# Autodesk Inventor assembly: ENSAMBLE_NUEVA_CREMALLERA
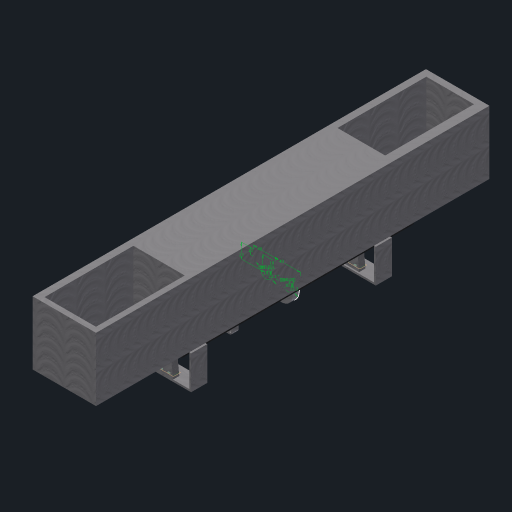
[picture p0: Inventor's stored thumbnail of the model, 512x512]
Saved by Autodesk Inventor 2024.3 (Build 283343000, 343)
## iProperties
Created: 2024-08-24
Part Number: ENSAMBLE_NUEVA_CREMALLERA
Material: Generic
Document SubType Name: Assembly
Designer: Niler
Author: Niler
## Documents named in this file (11)
- C:\Users\Niler\OneDrive\Escritorio\RECICLADOR\RECICLADOR_MODELO_3D\NUEVA CREMALLERA\ENSAMBLE_NUEVA_CREMALLERA.iam
- C:\Users\Niler\OneDrive\Escritorio\RECICLADOR\RECICLADOR_MODELO_3D\NUEVA CREMALLERA\TUBO.ipt
- C:\Users\Niler\OneDrive\Escritorio\RECICLADOR\RECICLADOR_MODELO_3D\NUEVA CREMALLERA\DESLIZANTE.ipt
- C:\Users\Niler\OneDrive\Escritorio\RECICLADOR\RECICLADOR_MODELO_3D\NUEVA CREMALLERA\APOYO_PLETINA.ipt
- C:\Users\Niler\OneDrive\Escritorio\RECICLADOR\RECICLADOR_MODELO_3D\NUEVA CREMALLERA\PARA_TUERCA.ipt
- C:\Users\Niler\OneDrive\Escritorio\RECICLADOR\RECICLADOR_MODELO_3D\NUEVA CREMALLERA\OTRO_EXTREMO.ipt
- C:\Users\Niler\OneDrive\Escritorio\RECICLADOR\RECICLADOR_MODELO_3D\NUEVA CREMALLERA\TORNILLO.ipt
- C:\Users\Niler\OneDrive\Escritorio\RECICLADOR\RECICLADOR_MODELO_3D\NUEVA CREMALLERA\GUIA.ipt
- C:\Users\Niler\OneDrive\Escritorio\RECICLADOR\RECICLADOR_MODELO_3D\MECANISMO DE COMPACTADO\NEMA 17 PARA TAPA PRINCIPAL.ipt
- C:\Users\Niler\OneDrive\Escritorio\RECICLADOR\RECICLADOR_MODELO_3D\MECANISMO DE COMPACTADO\ACOPLE_NEMA_PUERTA.ipt
- C:\Users\Niler\OneDrive\Escritorio\RECICLADOR\RECICLADOR_MODELO_3D\NUEVA CREMALLERA\PARA_TUERCA_V2.ipt
## Components (14 placed, 10 different names)
1. TUBO:1 — Flush:1, Mate:1, Mate:2, Mate:3, Mate:4, Mate:5
2. DESLIZANTE:1 — Flush:1, Mate:1, Flush:2, Mate:6, Mate:17
3. APOYO_PLETINA:1 — Mate:2, Mate:3, Mate:7, Flush:4, Mate:12, Flush:6, Mate:15
4. APOYO_PLETINA:2 — Mate:4, Mate:5, Mate:13
5. PARA_TUERCA:1 — Flush:2, Mate:6, Mate:8, Flush:5
6. OTRO_EXTREMO:1 — Mate:7, Flush:4, Mate:9, Mate:15
7. TORNILLO:1 — Mate:8, Mate:9, Mate:20, Mate:21
8. GUIA:1 — Mate:10, Mate:11, Mate:14, Mate:22
9. OTRO_EXTREMO:2 — Mate:10, Mate:12, Flush:6
10. OTRO_EXTREMO:3 — Mate:11, Mate:13
11. PARA_TUERCA:2 — Mate:14, Flush:5, Mate:17
12. NEMA 17 PARA TAPA PRINCIPAL:1 — Mate:20
13. ACOPLE_NEMA_PUERTA:1
14. PARA_TUERCA_V2:1 — Mate:21, Mate:22
## Relationships (27: Mate 21, Flush 5, Angle 1)
- Flush:1: TUBO:1 ↔ DESLIZANTE:1
- Mate:1: TUBO:1 ↔ DESLIZANTE:1
- Mate:2: TUBO:1 ↔ APOYO_PLETINA:1
- Mate:3: TUBO:1 ↔ APOYO_PLETINA:1
- Mate:4: TUBO:1 ↔ APOYO_PLETINA:2
- Mate:5: TUBO:1 ↔ APOYO_PLETINA:2
- Flush:2 (160 mm): DESLIZANTE:1 ↔ PARA_TUERCA:1
- Mate:6: DESLIZANTE:1 ↔ PARA_TUERCA:1
- Mate:7: APOYO_PLETINA:1 ↔ OTRO_EXTREMO:1
- Flush:4: APOYO_PLETINA:1 ↔ OTRO_EXTREMO:1
- Mate:8: PARA_TUERCA:1 ↔ TORNILLO:1
- Mate:9: OTRO_EXTREMO:1 ↔ TORNILLO:1
- Mate:10: GUIA:1 ↔ OTRO_EXTREMO:2
- Mate:11: GUIA:1 ↔ OTRO_EXTREMO:3
- Mate:12: APOYO_PLETINA:1 ↔ OTRO_EXTREMO:2
- Mate:13: APOYO_PLETINA:2 ↔ OTRO_EXTREMO:3
- Mate:14: GUIA:1 ↔ PARA_TUERCA:2
- Flush:5: PARA_TUERCA:1 ↔ PARA_TUERCA:2
- Flush:6: APOYO_PLETINA:1 ↔ OTRO_EXTREMO:2
- Mate:15 (15 mm): APOYO_PLETINA:1 ↔ OTRO_EXTREMO:1
- Mate:17: DESLIZANTE:1 ↔ PARA_TUERCA:2
- [Mate]: NEMA 17 PARA TAPA PRINCIPAL:1 ↔ ACOPLE_NEMA_PUERTA:1
- [Mate]: NEMA 17 PARA TAPA PRINCIPAL:1 ↔ ACOPLE_NEMA_PUERTA:1
- [Angle] (0 deg): NEMA 17 PARA TAPA PRINCIPAL:1 ↔ ACOPLE_NEMA_PUERTA:1
- Mate:20: TORNILLO:1 ↔ NEMA 17 PARA TAPA PRINCIPAL:1
- Mate:21: TORNILLO:1 ↔ PARA_TUERCA_V2:1
- Mate:22: GUIA:1 ↔ PARA_TUERCA_V2:1
